# Autodesk Inventor assembly: фуллл
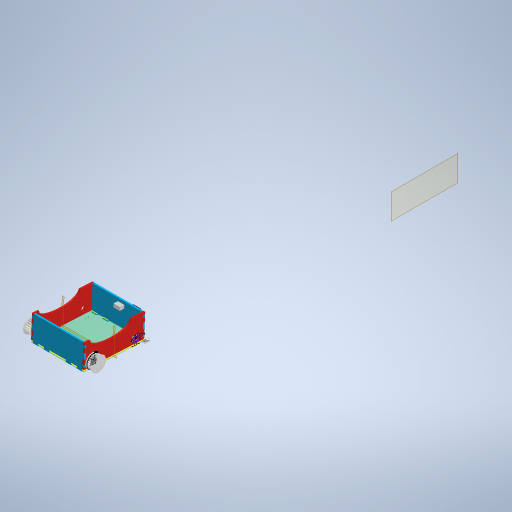
[picture p0: Inventor's stored thumbnail of the model, 512x512]
Saved by Autodesk Inventor 2024.2 (Build 282272000, 272)
## iProperties
Created: 2025-11-20
Part Number: фуллл
Document SubType Name: Assembly
Designer: Zakhar
Mass: 774.945 g
Surface Area: 2621.06 cm^2
Volume: 774.945 cm^3
Density: 1 g/cm^3
Author: Zakhar
## Documents named in this file (17)
- C:\Users\Zakhar\Documents\Artist\3D\Робот.iam
- C:\Users\Zakhar\Documents\Artist\3D\NEMA17 42-40.ipt
- C:\Users\Zakhar\Documents\Artist\3D\боковая стенка.ipt
- C:\Users\Zakhar\Documents\Artist\3D\Муфта.ipt
- C:\Users\Zakhar\Documents\Artist\3D\передняя стенка.ipt
- C:\Users\Zakhar\Documents\Artist\3D\Шест.ipt
- C:\Users\Zakhar\Documents\Artist\3D\Нижняя крышка.ipt
- C:\Users\Zakhar\Documents\Artist\3D\крепление подшипника_1.ipt
- C:\Users\Zakhar\Documents\Artist\3D\Муфта_MIR.ipt
- C:\Users\Zakhar\Documents\Artist\3D\Шест_MIR.ipt
- C:\Users\Zakhar\Documents\Artist\3D\полигон етз\полигон етз.ipt
- C:\Users\Zakhar\Documents\Artist\3D\робот-энкодер.ipt
- C:\Users\Zakhar\Documents\Artist\3D\для резинки.ipt
- C:\Users\Zakhar\Documents\Artist\3D\крутящаяся передача.ipt
- C:\Users\Zakhar\Documents\Artist\3D\стл\держатель вала.ipt
- C:\Users\Zakhar\Documents\Artist\3D\задняя стенка.ipt
- C:\Users\Zakhar\Documents\Artist\3D\каретка.iam
## Components (18 placed, 16 different names)
1. NEMA17 42-40:1 — Жесткий:5, С поворотом:2
2. боковая стенка:1 — Жесткий:12
3. Муфта:1 — С поворотом:1, Жесткий:8
4. Шест:1 — Жесткий:8, Заподлицо:1
5. боковая стенка:2 — Жесткий:5, Совмещение:2, Жесткий:10, Жесткий:11
6. Нижняя крышка:1 — Жесткий:10
7. NEMA17 42-40:2 — С поворотом:1
8. крепление подшипника_1:1
9. Муфта_MIR:1 — Жесткий:9, С поворотом:2
10. Шест_MIR:1 — Жесткий:9
11. полигон етз:1 — Совмещение:3, Заподлицо:1
12. робот-энкодер:1 — Совмещение:4, Совмещение:5, Совмещение:9, Совмещение:10
13. для резинки:1 — Совмещение:6, Совмещение:7, Совмещение:8
14. крутящаяся передача:1 — Совмещение:4, Совмещение:5, Совмещение:6, Совмещение:7, Совмещение:8
15. держатель вала:1
16. задняя стенка:1 — Жесткий:11, Жесткий:12, Совмещение:9, Совмещение:10, Совмещение:11, Совмещение:12, Совмещение:13
17. передняя стенка:1
18. каретка:1 [sub-assembly] — Совмещение:11, Совмещение:12, Совмещение:13
## Relationships (21: Mate 12, WeldJoint 6, RevoluteJoint 2, Flush 1)
- Жесткий:5 [WeldJoint]: NEMA17 42-40:1 ↔ боковая стенка:2
- Совмещение:2 [Mate]: боковая стенка:2
- С поворотом:1 [RevoluteJoint]: Муфта:1 ↔ NEMA17 42-40:2
- Жесткий:8 [WeldJoint]: Муфта:1 ↔ Шест:1
- Жесткий:9 [WeldJoint] (-4 mm): Муфта_MIR:1 ↔ Шест_MIR:1
- С поворотом:2 [RevoluteJoint]: NEMA17 42-40:1 ↔ Муфта_MIR:1
- Совмещение:3 [Mate] (-40.826 mm): полигон етз:1
- Заподлицо:1 [Flush] (4 mm): Шест:1 ↔ полигон етз:1
- Жесткий:10 [WeldJoint]: боковая стенка:2 ↔ Нижняя крышка:1
- Жесткий:11 [WeldJoint]: боковая стенка:2 ↔ задняя стенка:1
- Жесткий:12 [WeldJoint]: боковая стенка:1 ↔ задняя стенка:1
- Совмещение:4 [Mate]: робот-энкодер:1 ↔ крутящаяся передача:1
- Совмещение:5 [Mate]: робот-энкодер:1 ↔ крутящаяся передача:1
- Совмещение:6 [Mate]: для резинки:1 ↔ крутящаяся передача:1
- Совмещение:7 [Mate]: для резинки:1 ↔ крутящаяся передача:1
- Совмещение:8 [Mate]: для резинки:1 ↔ крутящаяся передача:1
- Совмещение:9 [Mate]: робот-энкодер:1 ↔ задняя стенка:1
- Совмещение:10 [Mate]: робот-энкодер:1 ↔ задняя стенка:1
- Совмещение:11 [Mate]: задняя стенка:1 ↔ каретка:1
- Совмещение:12 [Mate]: задняя стенка:1 ↔ каретка:1
- Совмещение:13 [Mate]: задняя стенка:1 ↔ каретка:1
